# Autodesk Inventor assembly: Drumstick
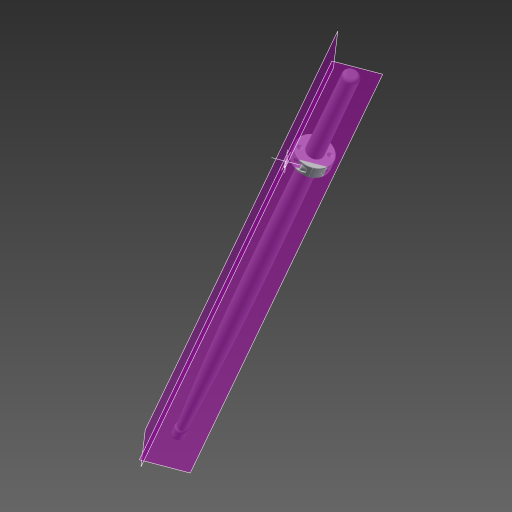
[picture p0: Inventor's stored thumbnail of the model, 512x512]
Saved by Autodesk Inventor 2023 (Build 270158000, 158)
## iProperties
Created: 2020-03-24
Part Number: Drumstick
Document SubType Name: Assembly
Designer: valer
Mass: 4853.13 g
Surface Area: 3141.52 cm^2
Volume: 1403.99 cm^3
Density: 3.45667 g/cm^3
Author: valer
## Documents named in this file (3)
- C:\Users\Val\Desktop\drummingrobot\src\parts\Drumstick.iam
- C:\Users\Val\Desktop\drummingrobot\src\parts\external\Drumstick.ipt
- C:\Users\Val\Desktop\drummingrobot\src\parts\external\ForearmShaftCollar.ipt
## Components (2 placed, 2 different names)
1. Drumstick:1 — Mate:79, Flush:3
2. ShaftCollar1/2:1 — Mate:79, Flush:3, Mate:80, Mate:81
## Relationships (4: Mate 3, Flush 1)
- Mate:79: Drumstick:1 ↔ ShaftCollar1/2:1
- Flush:3 (304.8 mm): Drumstick:1 ↔ ShaftCollar1/2:1
- Mate:80: ShaftCollar1/2:1
- Mate:81: ShaftCollar1/2:1
